# Autodesk Inventor assembly: Gear assembly
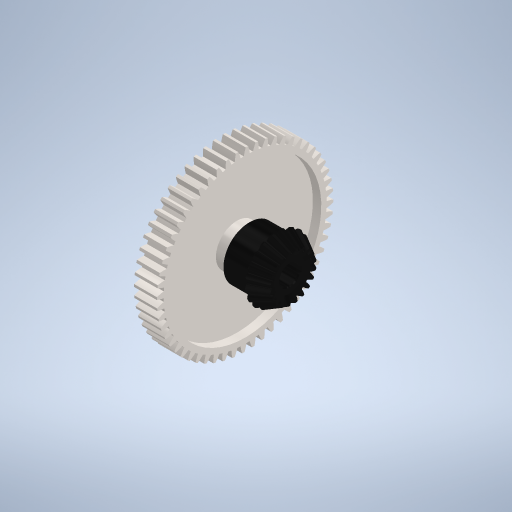
[picture p0: Inventor's stored thumbnail of the model, 512x512]
Saved by Autodesk Inventor 2023 (Build 270158000, 158)
## iProperties
Created: 2022-10-20
Part Number: Gear assembly
Document SubType Name: Assembly
Designer: cjj5381
Author: cjj5381
## Documents named in this file (3)
- C:\Users\Charles Kelly\Documents\Inventor\Robtooc\Apparatus\THE ARM\Gears\Gear assembly.iam
- C:\Users\Charles Kelly\Documents\Inventor\Robtooc\Apparatus\THE ARM\Gears\am-2621_20t_1-25mod_bevel_gear.ipt
- C:\Users\Charles Kelly\Documents\Inventor\Robtooc\Apparatus\THE ARM\Gears\am-3822 56T 20DP 500hex 375 FW.ipt
## Components (2 placed, 2 different names)
1. am-2621_20t_1-25mod_bevel_gear:1 — Mate:3, Mate:7
2. am-3822 56T 20DP 500hex 375 FW:1 — Mate:3, Mate:6, Mate:7
## Relationships (3: Mate 3)
- Mate:3: am-2621_20t_1-25mod_bevel_gear:1 ↔ am-3822 56T 20DP 500hex 375 FW:1
- Mate:6: am-3822 56T 20DP 500hex 375 FW:1
- Mate:7: am-2621_20t_1-25mod_bevel_gear:1 ↔ am-3822 56T 20DP 500hex 375 FW:1
